# Autodesk Inventor assembly: Minisumokokszloz
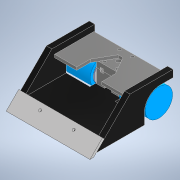
[picture p0: Inventor's stored thumbnail of the model, 180x180]
Saved by Autodesk Inventor 2022 (Build 260153000, 153)
## iProperties
Created: 2022-12-08
Part Number: Minisumokokszloz
Document SubType Name: Assembly
Designer: Kamil
Author: Kamil
## Documents named in this file (10)
- C:\MiniSumo koks\Minisumokokszloz.iam
- C:\MiniSumo koks\n20 motor.ipt
- C:\MiniSumo koks\felga.ipt
- C:\MiniSumo koks\opona.ipt
- C:\MiniSumo koks\Part8.ipt
- C:\MiniSumo koks\Part9.ipt
- C:\MiniSumo koks\lead.ipt
- C:\MiniSumo koks\nozyk.ipt
- C:\MiniSumo koks\uchwyt na plytke.ipt
- C:\MiniSumo koks\plugg.ipt
## Components (12 placed, 9 different names)
1. n20 motor:1 — Flush:1, Mate:1, Mate:2, Flush:8
2. n20 motor:2 — Flush:1, Mate:1, Mate:2, Flush:2, Flush:3, Flush:6, Flush:7
3. felga:1 — Flush:2, Flush:3
4. felga:2
5. opona:1
6. opona:2
7. Part8:1 — Flush:6, Flush:7, Flush:11
8. Part9:1 — Flush:8, Flush:9, Flush:10, Flush:13
9. lead:1 — Flush:9
10. nozyk:1 — Flush:10
11. uchwyt na plytke:1 — Flush:11
12. plugg:1 — Flush:13
## Relationships (12: Flush 10, Mate 2)
- Flush:1: n20 motor:1 ↔ n20 motor:2
- Mate:1 (5 mm): n20 motor:1 ↔ n20 motor:2
- Mate:2: n20 motor:1 ↔ n20 motor:2
- Flush:2: n20 motor:2 ↔ felga:1
- Flush:3: n20 motor:2 ↔ felga:1
- Flush:6: n20 motor:2 ↔ Part8:1
- Flush:7 (2.5 mm): n20 motor:2 ↔ Part8:1
- Flush:8: n20 motor:1 ↔ Part9:1
- Flush:9: Part9:1 ↔ lead:1
- Flush:10: Part9:1 ↔ nozyk:1
- Flush:11: Part8:1 ↔ uchwyt na plytke:1
- Flush:13: Part9:1 ↔ plugg:1
